# Autodesk Inventor assembly: Assembled Part
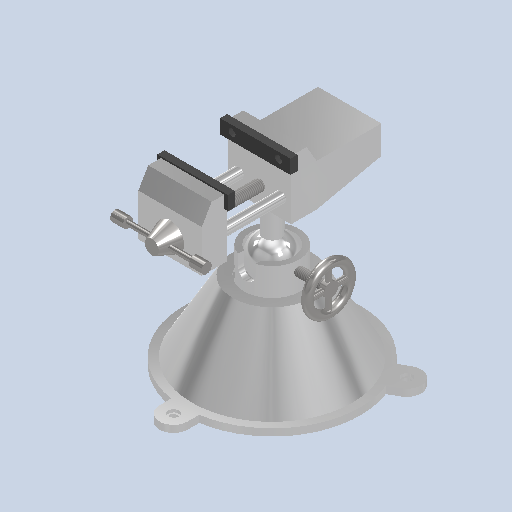
[picture p0: Inventor's stored thumbnail of the model, 512x512]
Saved by Autodesk Inventor 2024.3 (Build 283343000, 343)
## iProperties
Created: 2026-03-23
Part Number: Assembled Part
Document SubType Name: Assembly
Designer: Brett Morris
Project: Assembly
Description: Assembly Practice
Author: bam93065
## Documents named in this file (12)
- Z:\ENGR 1120 Graphic Design\Autodesk Inventor\Working Drawing Parts\Assembled Part.iam
- Z:\ENGR 1120 Graphic Design\Autodesk Inventor\Working Drawing Parts\P8-4b Base.ipt
- Z:\ENGR 1120 Graphic Design\Autodesk Inventor\Working Drawing Parts\P8-4c Casing.ipt
- Z:\ENGR 1120 Graphic Design\Autodesk Inventor\Working Drawing Parts\P8-4d Grip.ipt
- Z:\ENGR 1120 Graphic Design\Autodesk Inventor\Working Drawing Parts\P8-4e Head.ipt
- Z:\ENGR 1120 Graphic Design\Autodesk Inventor\Working Drawing Parts\P8-4f Jaw.ipt
- Z:\ENGR 1120 Graphic Design\Autodesk Inventor\Working Drawing Parts\P8-4g Pin.ipt
- Z:\ENGR 1120 Graphic Design\Autodesk Inventor\Working Drawing Parts\P8-4h Plate.ipt
- Z:\ENGR 1120 Graphic Design\Autodesk Inventor\Working Drawing Parts\P8-4i Shaft.ipt
- Z:\ENGR 1120 Graphic Design\Autodesk Inventor\Working Drawing Parts\P8-4j Wheel.ipt
- Z:\ENGR 1120 Graphic Design\Autodesk Inventor\Working Drawing Parts\ANSI B18.3 - 5-40 UNC - UNC - 0.25.ipt
- Z:\ENGR 1120 Graphic Design\Autodesk Inventor\Working Drawing Parts\ANSI B18.3 - 10-32 UNF - UNF - 0.3125.ipt
## Components (17 placed, 11 different names)
1. P8-4b Base:1 — Rigid:1, Rotational:1
2. P8-4c Casing:1 — Rigid:1, Mate:1, Mate:2, Mate:5
3. P8-4d Grip:1 — Rigid:3, Rigid:7, Rigid:8
4. P8-4e Head:1 — Mate:1, Mate:2, Mate:3, Mate:4, Angle:1, Angle:2, Rigid:2
5. P8-4f Jaw:1 — Mate:3, Mate:4, Rigid:3, Insert:1
6. P8-4g Pin:1 — Rigid:4
7. P8-4h Plate:1 — Rotational:1, Rotational:2, Rotational:3, Rigid:9
8. P8-4i Shaft:1 — Insert:1, Rigid:4
9. P8-4j Wheel:1 — Mate:5
10. P8-4d Grip:2 — Rigid:2, Rigid:5, Rigid:6
11. ANSI B18.3 - 5-40 UNC - UNC - 0.25:1 — Rigid:5
12. ANSI B18.3 - 5-40 UNC - UNC - 0.25:2 — Rigid:6
13. ANSI B18.3 - 5-40 UNC - UNC - 0.25:3 — Rigid:7
14. ANSI B18.3 - 5-40 UNC - UNC - 0.25:4 — Rigid:8
15. ANSI B18.3 - 10-32 UNF - UNF - 0.3125:1 — Rotational:2
16. ANSI B18.3 - 10-32 UNF - UNF - 0.3125:2 — Rotational:3
17. ANSI B18.3 - 10-32 UNF - UNF - 0.3125:3 — Rigid:9
## Relationships (20: WeldJoint 9, Mate 5, RevoluteJoint 3, Angle 2, Insert 1)
- Rigid:1 [WeldJoint]: P8-4b Base:1 ↔ P8-4c Casing:1
- Rotational:1 [RevoluteJoint]: P8-4b Base:1 ↔ P8-4h Plate:1
- Mate:1: P8-4c Casing:1 ↔ P8-4e Head:1
- Mate:2: P8-4c Casing:1 ↔ P8-4e Head:1
- Mate:3: P8-4e Head:1 ↔ P8-4f Jaw:1
- Mate:4: P8-4e Head:1 ↔ P8-4f Jaw:1
- Angle:1 (0 deg): P8-4e Head:1
- Angle:2 (0 deg): P8-4e Head:1
- Rigid:2 [WeldJoint]: P8-4e Head:1 ↔ P8-4d Grip:2
- Rigid:3 [WeldJoint]: P8-4d Grip:1 ↔ P8-4f Jaw:1
- Insert:1: P8-4f Jaw:1 ↔ P8-4i Shaft:1
- Mate:5: P8-4c Casing:1 ↔ P8-4j Wheel:1
- Rigid:4 [WeldJoint]: P8-4g Pin:1 ↔ P8-4i Shaft:1
- Rigid:5 [WeldJoint]: P8-4d Grip:2 ↔ ANSI B18.3 - 5-40 UNC - UNC - 0.25:1
- Rigid:6 [WeldJoint]: P8-4d Grip:2 ↔ ANSI B18.3 - 5-40 UNC - UNC - 0.25:2
- Rigid:7 [WeldJoint]: P8-4d Grip:1 ↔ ANSI B18.3 - 5-40 UNC - UNC - 0.25:3
- Rigid:8 [WeldJoint]: P8-4d Grip:1 ↔ ANSI B18.3 - 5-40 UNC - UNC - 0.25:4
- Rotational:2 [RevoluteJoint]: P8-4h Plate:1 ↔ ANSI B18.3 - 10-32 UNF - UNF - 0.3125:1
- Rotational:3 [RevoluteJoint]: P8-4h Plate:1 ↔ ANSI B18.3 - 10-32 UNF - UNF - 0.3125:2
- Rigid:9 [WeldJoint]: P8-4h Plate:1 ↔ ANSI B18.3 - 10-32 UNF - UNF - 0.3125:3
